# Autodesk Inventor assembly: RT_ARM_A_001
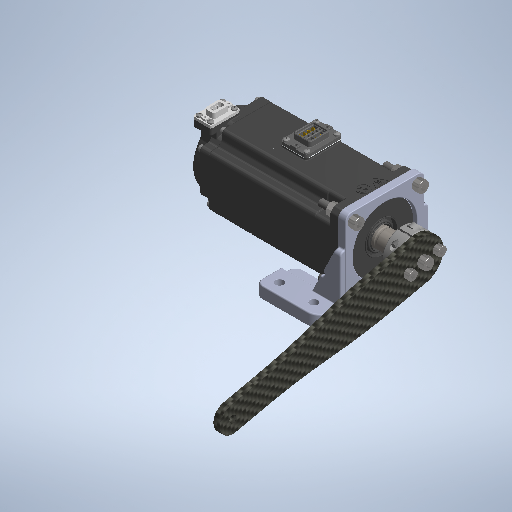
[picture p0: Inventor's stored thumbnail of the model, 512x512]
Saved by Autodesk Inventor 2025.4 (Build 294407000, 407)
## iProperties
Part Number: RT_ARM_A_001
Document SubType Name: Assembly
Designer: louis
Author: louis
## Documents named in this file (11)
- C:\Users\louis\OneDrive\Desktop\R_Trident\02_CAD\04_Subassemblies\RT_ARM_A_001.iam
- C:\Users\louis\OneDrive\Desktop\R_Trident\02_CAD\01_Standard_Parts\623 114 00GA\62311400GA.iam
- C:\Users\louis\OneDrive\Desktop\R_Trident\02_CAD\01_Standard_Parts\CFSTRIP-2-12-2.ipt
- C:\Users\louis\OneDrive\Desktop\R_Trident\02_CAD\03_Parts_Custom\RT_ARM_PR_001.ipt
- C:\Users\louis\OneDrive\Desktop\R_Trident\02_CAD\03_Parts_Custom\RT_ARM_MC_002.ipt
- C:\Users\louis\OneDrive\Desktop\R_Trident\02_CAD\01_Standard_Parts\A6M60-400H2B1-M17\A6M60-400H2B1-M17.iam
- C:\Users\louis\OneDrive\Documents\Inventor\Content Center Files\R2025\en-US\ISO 4762(2)\ISO 4762 - M4 x 6ISO.ipt
- C:\Users\louis\OneDrive\Documents\Inventor\Content Center Files\R2025\en-US\ISO 4762(2)\ISO 4762 - M5 x 8ISO.ipt
- C:\Users\louis\OneDrive\Desktop\R_Trident\02_CAD\01_Standard_Parts\ST-M4\ST-M4.ipt
- C:\Users\louis\OneDrive\Documents\Inventor\Content Center Files\R2025\en-US\ISO 4762(2)\ISO 4762 - M5 x 25ISO.ipt
- C:\Users\louis\OneDrive\Documents\Inventor\Content Center Files\R2025\en-US\ISO 4032(2)\ISO 4032 - M5 - ISO.ipt
## Components (18 placed, 10 different names)
1. 62311400GA:1 [sub-assembly] — Mate:1, Flush:3, Mate:4, Mate:5, Mate:6, Mate:7, Mate:9, Mate:11
2. CFSTRIP-2-12-2:1 — Mate:3
3. CFSTRIP-2-12-2:2 — Mate:2
4. RT_ARM_PR_001:1 — Mate:2, Mate:3, Mate:4
5. RT_ARM_MC_002:1 — Mate:5, Mate:6, Mate:8, Mate:10, Mate:12, Mate:14
6. A6M60-400H2B1-M17:1 [sub-assembly] — Mate:7, Mate:8, Mate:13, Mate:15, Mate:16, Mate:17, Insert:5, Insert:6, Insert:7, Insert:8
7. ISO 4762 M4 x 6:1 — Mate:9, Mate:10
8. ISO 4762 M4 x 6:2 — Mate:11, Mate:12
9. ISO 4762 M5 x 8:1 — Mate:13, Mate:14
10. ST-M4:1 — Mate:15, Mate:16, Mate:17, Mate:18, Insert:1, Insert:2, Insert:3, Insert:4
11. ISO 4762 M5 x 25:1 — Insert:1
12. ISO 4762 M5 x 25:2 — Insert:2
13. ISO 4762 M5 x 25:3 — Insert:3
14. ISO 4762 M5 x 25:4 — Insert:4
15. ISO 4032 M5:1 — Insert:5
16. ISO 4032 M5:2 — Insert:6
17. ISO 4032 M5:3 — Insert:7
18. ISO 4032 M5:4 — Insert:8
## Relationships (27: Mate 18, Insert 8, Flush 1)
- Mate:1: 62311400GA:1
- Flush:3: 62311400GA:1
- Mate:2: CFSTRIP-2-12-2:2 ↔ RT_ARM_PR_001:1
- Mate:3: CFSTRIP-2-12-2:1 ↔ RT_ARM_PR_001:1
- Mate:4: 62311400GA:1 ↔ RT_ARM_PR_001:1
- Mate:5: 62311400GA:1 ↔ RT_ARM_MC_002:1
- Mate:6: 62311400GA:1 ↔ RT_ARM_MC_002:1
- Mate:7: 62311400GA:1 ↔ A6M60-400H2B1-M17:1
- Mate:8: RT_ARM_MC_002:1 ↔ A6M60-400H2B1-M17:1
- Mate:9: 62311400GA:1 ↔ ISO 4762 M4 x 6:1
- Mate:10: RT_ARM_MC_002:1 ↔ ISO 4762 M4 x 6:1
- Mate:11: 62311400GA:1 ↔ ISO 4762 M4 x 6:2
- Mate:12: RT_ARM_MC_002:1 ↔ ISO 4762 M4 x 6:2
- Mate:13: A6M60-400H2B1-M17:1 ↔ ISO 4762 M5 x 8:1
- Mate:14: RT_ARM_MC_002:1 ↔ ISO 4762 M5 x 8:1
- Mate:15: A6M60-400H2B1-M17:1 ↔ ST-M4:1
- Mate:16: A6M60-400H2B1-M17:1 ↔ ST-M4:1
- Mate:17: A6M60-400H2B1-M17:1 ↔ ST-M4:1
- Mate:18: ST-M4:1
- Insert:1: ST-M4:1 ↔ ISO 4762 M5 x 25:1
- Insert:2: ST-M4:1 ↔ ISO 4762 M5 x 25:2
- Insert:3: ST-M4:1 ↔ ISO 4762 M5 x 25:3
- Insert:4: ST-M4:1 ↔ ISO 4762 M5 x 25:4
- Insert:5: A6M60-400H2B1-M17:1 ↔ ISO 4032 M5:1
- Insert:6: A6M60-400H2B1-M17:1 ↔ ISO 4032 M5:2
- Insert:7: A6M60-400H2B1-M17:1 ↔ ISO 4032 M5:3
- Insert:8: A6M60-400H2B1-M17:1 ↔ ISO 4032 M5:4
